# Autodesk Inventor assembly: TestAssm
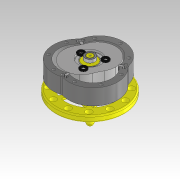
[picture p0: Inventor's stored thumbnail of the model, 180x180]
Saved by Autodesk Inventor 2020 (Build 240168000, 168)
## iProperties
Created: 2021-05-17
Part Number: TestAssm
Document SubType Name: Assembly
Designer: DDeGo
Author: DDeGo
## Documents named in this file (19)
- C:\Users\DDeGo\Documents\Drew\Projects\AirWankelEngine\cad\LiquidPiston V1.6\TestAssm.iam
- C:\Users\DDeGo\Documents\Drew\Projects\AirWankelEngine\cad\LiquidPiston V1.6\Housing.ipt
- C:\Users\DDeGo\Documents\Drew\Projects\AirWankelEngine\cad\LiquidPiston V1.6\CamThing.ipt
- C:\Users\DDeGo\Documents\Drew\Projects\AirWankelEngine\cad\LiquidPiston V1.6\TestAssm\Design Accelerator\Spur Gears1.iam
- C:\Users\DDeGo\Documents\Drew\Projects\AirWankelEngine\cad\hardware\6701 bearing.ipt
- C:\Users\DDeGo\Documents\Drew\Projects\AirWankelEngine\cad\LiquidPiston V1.6\Head.ipt
- C:\Users\DDeGo\Documents\Drew\Projects\AirWankelEngine\cad\LiquidPiston V1.6\ApexSeal.ipt
- C:\Users\DDeGo\Documents\Drew\Projects\AirWankelEngine\cad\hardware\MR85 bearing.ipt
- C:\Users\DDeGo\Documents\Drew\Projects\AirWankelEngine\cad\LiquidPiston V1.6\Flywheel.ipt
- C:\Users\DDeGo\Documents\Drew\Projects\AirWankelEngine\cad\hardware\2x22 pin.ipt
- C:\Users\DDeGo\Documents\Drew\Projects\AirWankelEngine\cad\LiquidPiston V1.6\FlywheelXL.ipt
- C:\Users\DDeGo\Documents\Drew\Projects\AirWankelEngine\cad\LiquidPiston V1.6\MotorTestBracket.ipt
- C:\Users\DDeGo\Documents\Drew\Projects\AirWankelEngine\cad\LiquidPiston V1.6\2020 Extrusion.ipt
- C:\Users\DDeGo\Documents\Drew\Projects\AirWankelEngine\cad\LiquidPiston V1.6\TestLever.ipt
- C:\Users\DDeGo\Documents\Drew\Projects\AirWankelEngine\cad\LiquidPiston V1.6\TestEncoderBracket.ipt
- C:\Users\DDeGo\Documents\Drew\Projects\AirWankelEngine\cad\LiquidPiston V1.6\TestEncoder.ipt
- C:\Users\DDeGo\Documents\Drew\Projects\AirWankelEngine\cad\hardware\oring_2x6.ipt
- C:\Users\DDeGo\Documents\Drew\Projects\AirWankelEngine\cad\LiquidPiston V1.6\Rotor_NEW.ipt
- C:\Users\DDeGo\Documents\Drew\Projects\AirWankelEngine\cad\LiquidPiston V1.6\TestAssm\Design Accelerator\Spur Gears2.iam
## Components (23 placed, 17 different names)
1. Housing:1 — Mate:11, Mate:14, Mate:15, Mate:20, Mate:21, Mate:66, Mate:67, Mate:68, Mate:69, Mate:80, Flush:7, Mate:105
2. CamThing:1 — Flush:6, Mate:94, Mate:98, Mate:104, Rotation:1, Flush:11, Angle:3
3. Spur Gears:1 [sub-assembly]
4. 6701 bearing:1 — Flush:6, Mate:104, Mate:106, Mate:107
5. ApexSeal:1 — Mate:11, Mate:67
6. ApexSeal:2 — Mate:14, Mate:68
7. ApexSeal:3 — Mate:15, Mate:66
8. MR85 bearing:1 — Mate:20, Mate:21, Mate:32, Mate:33
9. MR85 bearing:2 — Mate:64, Mate:95, Mate:98
10. Flywheel:1 — Mate:32, Mate:33, Mate:45, Mate:77, Mate:79, Angle:3
11. 2x22 pin:1 — Mate:45, Mate:78, Mate:94, Flush:11
12. Head:1 — Mate:64, Mate:69, Mate:95, Mate:100, Mate:101, Mate:102, Tangent:1, Tangent:2, Tangent:3
13. FlywheelXL:1 — Mate:77, Mate:78, Mate:79, Mate:83, Mate:84, Mate:93, Angle:2
14. MotorTestBracket:1 — Mate:80, Flush:7, Mate:82, Flush:8, Flush:9
15. 2020 Extrusion:1 — Mate:82, Flush:8, Flush:9, Mate:89, Flush:10
16. TestLever:1 — Mate:83, Mate:84
17. TestEncoderBracket:1 — Mate:89, Flush:10, Mate:90, Mate:91, Mate:92
18. TestEncoder:1 — Mate:90, Mate:91, Mate:92, Mate:93
19. oring_2x6:1 — Mate:101, Tangent:1
20. oring_2x6:2 — Mate:100, Tangent:3
21. oring_2x6:3 — Mate:102, Tangent:2
22. Rotor_NEW:1 — Mate:105, Mate:106, Mate:107, Rotation:1
23. Spur Gears:2 [sub-assembly]
## Relationships (47: Mate 35, Flush 6, Tangent 3, Angle 2, RelateRotation 1)
- Mate:11 (0.1 mm): Housing:1 ↔ ApexSeal:1
- Mate:14 (0.1 mm): Housing:1 ↔ ApexSeal:2
- Mate:15 (0.1 mm): Housing:1 ↔ ApexSeal:3
- Mate:20: Housing:1 ↔ MR85 bearing:1
- Mate:21: Housing:1 ↔ MR85 bearing:1
- Mate:32: MR85 bearing:1 ↔ Flywheel:1
- Mate:33: MR85 bearing:1 ↔ Flywheel:1
- Mate:45: Flywheel:1 ↔ 2x22 pin:1
- Flush:6: CamThing:1 ↔ 6701 bearing:1
- Mate:64: MR85 bearing:2 ↔ Head:1
- Mate:66: Housing:1 ↔ ApexSeal:3
- Mate:67: Housing:1 ↔ ApexSeal:1
- Mate:68: Housing:1 ↔ ApexSeal:2
- Mate:69 (0.2 mm): Housing:1 ↔ Head:1
- Mate:77: Flywheel:1 ↔ FlywheelXL:1
- Mate:78: 2x22 pin:1 ↔ FlywheelXL:1
- Mate:79: Flywheel:1 ↔ FlywheelXL:1
- Mate:80: Housing:1 ↔ MotorTestBracket:1
- Flush:7 (-1 mm): Housing:1 ↔ MotorTestBracket:1
- Mate:82: MotorTestBracket:1 ↔ 2020 Extrusion:1
- Flush:8: MotorTestBracket:1 ↔ 2020 Extrusion:1
- Flush:9 (5 mm): MotorTestBracket:1 ↔ 2020 Extrusion:1
- Mate:83: FlywheelXL:1 ↔ TestLever:1
- Mate:84: FlywheelXL:1 ↔ TestLever:1
- Mate:89: 2020 Extrusion:1 ↔ TestEncoderBracket:1
- Flush:10: 2020 Extrusion:1 ↔ TestEncoderBracket:1
- Mate:90: TestEncoderBracket:1 ↔ TestEncoder:1
- Mate:91: TestEncoderBracket:1 ↔ TestEncoder:1
- Mate:92: TestEncoderBracket:1 ↔ TestEncoder:1
- Mate:93: FlywheelXL:1 ↔ TestEncoder:1
- Mate:94: CamThing:1 ↔ 2x22 pin:1
- Mate:95: MR85 bearing:2 ↔ Head:1
- Mate:98: CamThing:1 ↔ MR85 bearing:2
- Mate:100: Head:1 ↔ oring_2x6:2
- Mate:101: Head:1 ↔ oring_2x6:1
- Mate:102: Head:1 ↔ oring_2x6:3
- Tangent:1: Head:1 ↔ oring_2x6:1
- Tangent:2: Head:1 ↔ oring_2x6:3
- Tangent:3: Head:1 ↔ oring_2x6:2
- Mate:104: CamThing:1 ↔ 6701 bearing:1
- Angle:2 (0 deg): FlywheelXL:1
- Mate:105: Housing:1 ↔ Rotor_NEW:1
- Mate:106: 6701 bearing:1 ↔ Rotor_NEW:1
- Mate:107: 6701 bearing:1 ↔ Rotor_NEW:1
- Rotation:1 [RelateRotation] (0.5 ul): CamThing:1 ↔ Rotor_NEW:1
- Flush:11 (-0.5 mm): CamThing:1 ↔ 2x22 pin:1
- Angle:3 (180 deg): CamThing:1 ↔ Flywheel:1
